# Autodesk Inventor assembly: axle wheel
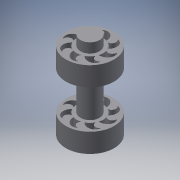
[picture p0: Inventor's stored thumbnail of the model, 180x180]
Saved by Autodesk Inventor 2018 (Build 220112000, 112)
## iProperties
Created: 2020-01-09
Part Number: axle wheel
Document SubType Name: Assembly
Designer: AOFUser
Author: AOFUser
## Documents named in this file (3)
- C:\Users\AOFUser\Desktop\Park_CAD\axle wheel.iam
- C:\Users\AOFUser\Desktop\Park_CAD\axle.ipt
- C:\Users\AOFUser\Desktop\Park_CAD\whee.ipt
## Components (3 placed, 2 different names)
1. axle:1 — Mate:1, Mate:2, Flush:1, Flush:2
2. whee:1 — Mate:2, Flush:1
3. whee:2 — Mate:1, Flush:2
## Relationships (4: Mate 2, Flush 2)
- Mate:1: axle:1 ↔ whee:2
- Mate:2: axle:1 ↔ whee:1
- Flush:1 (12.7 mm): axle:1 ↔ whee:1
- Flush:2 (12.7 mm): axle:1 ↔ whee:2
